# Autodesk Inventor assembly: Động cơ 775 + Giảm tốc
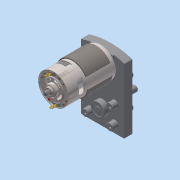
[picture p0: Inventor's stored thumbnail of the model, 180x180]
Saved by Autodesk Inventor 2018 (Build 220112000, 112)
## iProperties
Created: 2020-10-09
Part Number: Động cơ 775 + Giảm tốc
Document SubType Name: Assembly
Designer: ASUS
Author: ASUS
## Documents named in this file (3)
- E:\CTU\Skylight\Bản vẽ\Bản vẽ Giếng Trời Tự Động\Bản vẽ 3D\Động cơ 775 + Giảm tốc\Động cơ 775 + Giảm tốc.iam
- E:\CTU\Skylight\Bản vẽ\Bản vẽ Giếng Trời Tự Động\Bản vẽ 3D\Động cơ 775 + Giảm tốc\Giảm tốc DC 775.ipt
- E:\CTU\Skylight\Bản vẽ\Bản vẽ Giếng Trời Tự Động\Bản vẽ 3D\Động cơ 775 + Giảm tốc\Motor - RS-775.ipt
## Components (2 placed, 2 different names)
1. Giảm tốc DC 775:1 — Mate:1, Mate:2
2. Motor - RS-775:1 — Mate:1, Mate:2
## Relationships (2: Mate 2)
- Mate:1: Giảm tốc DC 775:1 ↔ Motor - RS-775:1
- Mate:2: Giảm tốc DC 775:1 ↔ Motor - RS-775:1
